# Autodesk Inventor assembly: Rack Assembly
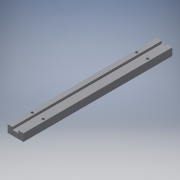
[picture p0: Inventor's stored thumbnail of the model, 180x180]
Saved by Autodesk Inventor 2016 (Build 200138000, 138)
## iProperties
Created: 2016-04-12
Part Number: Rack Assembly
Document SubType Name: Assembly
Designer: Andrea
Author: Andrea
## Documents named in this file (3)
- C:\Users\Andrea\Documents\Dropbox\Capstone CAD\Rack Assembly.iam
- C:\Users\Andrea\Documents\Dropbox\Capstone CAD\Rack Bottom.ipt
- C:\Users\Andrea\Documents\Dropbox\Capstone CAD\Rack Side.ipt
## Components (3 placed, 2 different names)
1. Rack Bottom:1 — Mate:1, Mate:2, Mate:3, Mate:4, Mate:5, Mate:6, Mate:7, Mate:8, Mate:9, Mate:10
2. Rack Side:1 — Mate:1, Mate:2, Mate:5, Mate:6, Mate:7
3. Rack Side:2 — Mate:3, Mate:4, Mate:8, Mate:9, Mate:10
## Relationships (10: Mate 10)
- Mate:1: Rack Bottom:1 ↔ Rack Side:1
- Mate:2: Rack Bottom:1 ↔ Rack Side:1
- Mate:3: Rack Bottom:1 ↔ Rack Side:2
- Mate:4: Rack Bottom:1 ↔ Rack Side:2
- Mate:5: Rack Bottom:1 ↔ Rack Side:1
- Mate:6: Rack Bottom:1 ↔ Rack Side:1
- Mate:7: Rack Bottom:1 ↔ Rack Side:1
- Mate:8: Rack Bottom:1 ↔ Rack Side:2
- Mate:9: Rack Bottom:1 ↔ Rack Side:2
- Mate:10: Rack Bottom:1 ↔ Rack Side:2
